# Autodesk Inventor assembly: head_mind_long_side
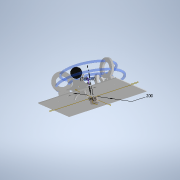
[picture p0: Inventor's stored thumbnail of the model, 180x180]
Saved by Autodesk Inventor 2021.1 (Build 251245010, 245A)
## iProperties
Created: 2022-11-16
Part Number: head_mind_long_side
Document SubType Name: Assembly
Designer: zmoze
Author: zmoze
## Documents named in this file (8)
- C:\Users\zmoze\OneDrive\Рабочий стол\GrabCAD\Smile_2022-2023\head_mind_long_side.iam
- C:\Users\zmoze\OneDrive\Рабочий стол\GrabCAD\Smile_2022-2023\панель_электроники_и не только.ipt
- C:\Users\zmoze\OneDrive\Рабочий стол\GrabCAD\Smile_2022-2023\шаговый_мотор.ipt
- C:\Users\zmoze\OneDrive\Рабочий стол\GrabCAD\Smile_2022-2023\шестеренка_для_мозговорота.ipt
- C:\Users\zmoze\OneDrive\Рабочий стол\GrabCAD\Smile_2022-2023\держалка_мозговорота.iam
- C:\Users\zmoze\OneDrive\Рабочий стол\GrabCAD\Smile_2022-2023\трубочки_мозговорота.ipt
- C:\Users\zmoze\OneDrive\Рабочий стол\GrabCAD\Smile_2022-2023\мячик_для_тенниса.ipt
- C:\Users\zmoze\OneDrive\Рабочий стол\GrabCAD\Smile_2022-2023\крепление_мотора_для_шестерни.iam
## Components (9 placed, 7 different names)
1. панель_электроники_и не только:1 — Совмещение:6, Совмещение:7, Совмещение:8, Совмещение:14, Совмещение:15, Заподлицо:1, Совмещение:16, Совмещение:17, Совмещение:18, Заподлицо:2
2. шестеренка_для_мозговорота:1 — Совмещение:19, Заподлицо:2, Совмещение:20
3. трубочки_мозговорота:1 — Совмещение:14, Касательность:4, Касательность:5, Касательность:6, Обкатка:1, Обкатка:2, Обкатка:3
4. мячик_для_тенниса:1 — Обкатка:1, Обкатка:2, Обкатка:3
5. шаговый_мотор:1 — Совмещение:15, Заподлицо:1, Совмещение:16
6. крепление_мотора_для_шестерни:1 [sub-assembly] — Совмещение:17, Совмещение:18, Совмещение:19, Совмещение:20
7. держалка_мозговорота:1 [sub-assembly] — Совмещение:6, Совмещение:7, Совмещение:8, Касательность:4, Касательность:5, Касательность:6
8. держалка_мозговорота:2 [sub-assembly]
9. держалка_мозговорота:3 [sub-assembly]
## Component patterns: (3 elements, first: держалка_мозговорота:1)
## Relationships (18: Mate 10, Tangent 3, Transitional 3, Flush 2)
- Совмещение:6 [Mate]: панель_электроники_и не только:1 ↔ держалка_мозговорота:1
- Совмещение:7 [Mate]: панель_электроники_и не только:1 ↔ держалка_мозговорота:1
- Совмещение:8 [Mate] (90 mm): панель_электроники_и не только:1 ↔ держалка_мозговорота:1
- Совмещение:14 [Mate]: панель_электроники_и не только:1 ↔ трубочки_мозговорота:1
- Совмещение:15 [Mate]: панель_электроники_и не только:1 ↔ шаговый_мотор:1
- Заподлицо:1 [Flush]: панель_электроники_и не только:1 ↔ шаговый_мотор:1
- Совмещение:16 [Mate]: панель_электроники_и не только:1 ↔ шаговый_мотор:1
- Касательность:4 [Tangent]: трубочки_мозговорота:1 ↔ держалка_мозговорота:1
- Касательность:5 [Tangent]: трубочки_мозговорота:1 ↔ держалка_мозговорота:1
- Касательность:6 [Tangent]: трубочки_мозговорота:1 ↔ держалка_мозговорота:1
- Обкатка:1 [Transitional]: трубочки_мозговорота:1 ↔ мячик_для_тенниса:1
- Обкатка:2 [Transitional]: трубочки_мозговорота:1 ↔ мячик_для_тенниса:1
- Обкатка:3 [Transitional]: трубочки_мозговорота:1 ↔ мячик_для_тенниса:1
- Совмещение:17 [Mate]: панель_электроники_и не только:1 ↔ крепление_мотора_для_шестерни:1
- Совмещение:18 [Mate] (10 mm): панель_электроники_и не только:1 ↔ крепление_мотора_для_шестерни:1
- Совмещение:19 [Mate]: шестеренка_для_мозговорота:1 ↔ крепление_мотора_для_шестерни:1
- Заподлицо:2 [Flush] (94 mm): панель_электроники_и не только:1 ↔ шестеренка_для_мозговорота:1
- Совмещение:20 [Mate]: шестеренка_для_мозговорота:1 ↔ крепление_мотора_для_шестерни:1
